# Autodesk Inventor assembly: SR-092.5-DPY
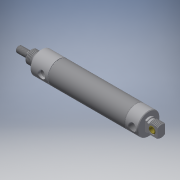
[picture p0: Inventor's stored thumbnail of the model, 180x180]
Saved by Autodesk Inventor 2016 SP1 (Build 200210100, 210)
## iProperties
Category: PARTsolutions
Company: BIMBA
Created: 2017-03-09
Part Number: SR-092.5-DPY
Catalog Web Link: www.cadenas.de
Description: Original Line Standard Air Cylinders-
Vendor: BIMBA
Document SubType Name: Assembly
Designer: 589013
Manufacturer: BIMBA
PSOL_IDENT_0: {$CADENAS_DATA\23d-libs\bimba\bimba\bimba_imperial\bimba_full_line\original_line_cylinders\standard_
PSOL_IDENT_1: air_cylinders\standard_air_cylinder_asmtab.prj},324 {VTYP=3D},{STYP=ASSTAB},{NB=SR-092.5-DPY},{LINA=
PSOL_IDENT_2: SR-092.5-DPY},{NN=Original Line Standard Air Cylinders},{DATE=09.11.2016 07:55:11},{GEOMDATE=11.07.2
PSOL_IDENT_3: 016 10:37:18},{VERSION=},{LINEID=10},{LINESUBID=-1},{WBVAR=STROKE,ACTING,MNT,DER,NR,BM,CO,OO,VO,M,EE
PSOL_IDENT_4: ,EEL,K,Q,Y,G,T,B,H,SER,SR,NT,W,HL,STPT1,STPT2,STPT3,STPT4,MB,PB,PRC,TB,MN}  {NB=SR-092.5-DPY},{LINA=
PSOL_IDENT_5: SR-092.5-DPY},{KT=DUMMY},{PN=SR-092.5-DPY},{PNC=SR-092.5-DPY},{PNA=(NO ACCESSORIES)},{DASH=-},{BORE1=
PSOL_IDENT_6: 1.06250000},{BORE=1 1/16\" (09)},{BOREPN=09},{STROKE=2.500},{STROKEALG=[0.011:50/0.001]},{STROKE1=2.
PSOL_IDENT_7: 500},{ACTING=D},{ACTINGALG= '' , 'Single Acting (SA)' , 'R' , 'Reverse Single Acting (SA)' , 'D' , '
PSOL_IDENT_8: Double Acting (SA)' },{ACTINGPN=D},{MNT=P},{MNTALG= '' , 'Front Nose Mounting (SA)' , 'P' , 'Rear Pi
PSOL_IDENT_9: vot Mounting (SA)' , 'X' , 'Universal Pivot Mounting or Double End Mounting (SA)' , 'BF' , 'Front Bl
PSOL_IDENT_10: ock Mounting (SA)' , 'BR' , 'Rear Block Mounting for Vertical Positioning (SA)' , 'BFT' , 'Front Blo
PSOL_IDENT_11: ck Trunnion Mounting (SA)' , 'BRT' , 'Rear Block Trunnion Mounting (SA)' },{TYPE=SR-},{MNTPN=P},{DER=
PSOL_IDENT_12: },{DERALG= '' , 'N/A' },{NR=},{NRALG= '' , 'N/A' },{NRPN=},{BM=},{BMALG= '' , 'N/A' },{BMPN=},{CO=},
PSOL_IDENT_13: {COALG= '' , 'N/A' },{OO=},{OOALG= '', 'N/A' },{OOPN=},{VO=Z},{VOALG= 'Z' , 'N/A' },{VOPN=},{OOVOPN=
PSOL_IDENT_14: },{M=},{MALG= '', 'Without Magnet', 'M', 'With Magnet' },{EE=},{EEL=0.000},{EEMAX=47.5000},{EEALG= ''
PSOL_IDENT_15: , 'Without Extra Extension', 'EE', 'With Extra Extension' },{EELALG=0},{EEPN=},{EEPN1=0.000},{K=},{K
PSOL_IDENT_16: ALG= '', 'Standard' , 'K' , 'Ports Rotated 90deg K' },{KPN=},{Q=},{QALG= '' , 'N/A' },{QPN=},{Y=Y},{
PSOL_IDENT_17: YALG= '' , 'Without Pivot Bushing' , 'Y' , 'With Pivot Bushing' },{YPN=Y},{YCON=Y},{F=},{FALG= '', '
PSOL_IDENT_18: Non-Coated (Standard)', 'F', 'Molycoated' },{FPN=},{G=},{GPN=},{GPN99=},{T=},{TALG= '' , 'Standard -
PSOL_IDENT_19: 20° to 200°F (-29° to 95°C)' , 'N' , 'Low Temperature' , 'V' , 'High Temperature' },{NPN=},{VPN=},{B=
PSOL_IDENT_20: },{BALG= '', 'W/out Bumpers' , 'B' , 'W/ Bumpers' },{BPN=},{H=},{HALG= '', 'N/A' },{HPN=},{SER=},{SE
PSOL_IDENT_21: RALG= '' , 'Without Spring Extend/Return' , 'JS' , 'With Spring Return' , 'JR' , 'With Spring Extend'
PSOL_IDENT_22: },{SR=SR},{SRALG= 'C' , 'Standard Blackened Carbon Steel' , 'SR' , 'Stainless Steel [SR]' },{SRPN=S
PSOL_IDENT_23: R},{SRCON=1},{NT=},{NTPN=},{W=},{WALG= '' , 'Without Wiper' , 'W' , 'With Wiper' },{WPN=},{E=},{EALG=
PSOL_IDENT_24: '' , 'Standard Seals/Lube' , 'E' , 'Non-Lube Seals/Lube' },{EPN=},{HL=},{HLALG= '' , 'Without Low P
PSOL_IDENT_25: ressure Hydraulic' , 'HL' , 'With Low Pressure Hydraulic' },{ST=},{STALG= '' , 'N/A' },{STPT1=},{STP
PSOL_IDENT_26: T1ALG= '' , 'N/A' },{STPT2=},{STPT2ALG= '' , 'N/A' },{STPT3=},{STPT3ALG= '' , 'N/A' },{STPT4=},{STPT
PSOL_IDENT_27: 4ALG= '' , 'N/A' },{STPN=},{MB=},{MBALG= '' , 'N/A' },{MBPN=},{MBPNALL=},{MBPNALLREAR=},{PB=},{PBALG=
PSOL_IDENT_28: '' , 'Without Pivot Bracket' , 'D-13498-A' , 'D-13498-A' },{PBPN=},{PBPNALL=D-13498-A},{PRC=},{PRCA
PSOL_IDENT_29: LG= '' , 'W/out Pivot Rod Clevis' , 'F,D-166-1' , 'D-166-1 (front)' },{PRCPN=},{PRCPNALL=D-166-1},{T
PSOL_IDENT_30: B=},{TBALG= '' , 'N/A' },{TBPN=},{TBPNALL=},{MN=},{MNALG= '' , 'Without Mounting Nut' , 'F,D-9' , 'D
PSOL_IDENT_31: -9 (front)' , 'R,D-9' , 'D-9 (rear)', '2x,D-9' , 'D-9 (front & rear)' },{MNPN=},{MNCONF=},{MNCONR=},
PSOL_IDENT_32: {TLEN=3.8185},{FRAC=10.8400},{RGCON=},{RGDACCON=R},{RHCON=P},{RHCON1=P},{RHCONON=1},{RHACCON=},{FNUT
PSOL_IDENT_33: CON=0},{RNUTCON=0},{FNUTPN=D-9},{RNUTPN=D-9},{FNUTTRANS=0.0000},{RNUTTRANS=0.0000},{VHOLECON=0},{A1=
PSOL_IDENT_34: 1.6250},{A1N=1.0000},{A1P=1.6250},{A1B=1.8750},{A4=0.2525},{A4N=0.3750},{A4P=0.2525},{A5=0.0300},{A1
PSOL_IDENT_35: H=1.5},{A1NH=0.6250},{A1PH=1.5000},{A1BH=1.1250},{A1SH=1.1250},{A2H=0.2500},{A2NH=0.2500},{LENGTH=3.
PSOL_IDENT_36: 8400},{LENGTH1=3.8400},{LENGTH2=4.1000},{MUL=2.5000},{MUL11=2.5000},{MUL22=6.4},{MUL33=3.9000},{MUL2=
PSOL_IDENT_37: 2.5000},{MUL211=2.5000},{MUL222=2.5600},{MUL233=1.5600},{SSS=5.0000},{RGLEN=1.4025},{RHLEN=0.9990},{
PSOL_IDENT_38: SSS1=3.0000},{A13=1.2190},{DIF=0.1200},{G5=0.7180},{ON=0},{SSADD=0.0000},{BADD=0.0000},{MADD=0.0000}
PSOL_IDENT_39: ,{NVADD=0.0000},{TRACKL=3.5285},{TRACKCON=D-78527},{TRIMCON=0},{TRIMCON1=0},{PINCON=},{FSPACE=0.7678
PSOL_IDENT_40: },{SPACE=0.0987},{TEXT=0.1727},{S1=1.2500},{D1=1.1410},{D1N=1.1130},{D1B=1.1130},{D1P=1.1410},{FA=0.
PSOL_IDENT_41: 940},{RA=0.9400},{PPATH=standard_air_cylinder_asmtpl.prj},{MATALGHTML=<b>Standard Original Line:</b>
PSOL_IDENT_42: <dl><dt>Rod:</dt><dd>- Stainless Steel</dd><dd>&nbsp;&nbsp;(5/16 9/16 Bores)</dd><dd>- High Strength
PSOL_IDENT_43: Carbon Steel</dd><dd>&nbsp;&nbsp;(3/4 3 Bore)</dd><dd>- Stainless Steel</dd><dd>&nbsp;&nbsp;(X styl
PSOL_IDENT_44: e DXP/DX/DXDE)</dd><dt>Bearings:</dt><dd>- Sintered Bronze</dd><dt>Body:</dt><dd>- 304 Stainless Ste
PSOL_IDENT_45: el</dd><dt>End Caps:</dt><dd>- Aluminum</dd><dt>Seals:</dt><dd>- Buna N</dd></dl>},{ASSCFGPRA=09DP},
PSOL_IDENT_46: {MBPNA=},{MNPNA=},{PRCPNA=},{ASSOPTACC=STPT4},{A=6.34},{HADD=0.0000},{WFL=0.125},{QADD=0.000},{QADD1=
PSOL_IDENT_47: 0.250},{TEST=2.0000},{MNTB=},{STDNUTF=0},{STDNUTR=0},{STRK2D=0},{X2D=2},{STROKESW=2.500},{EESW=0.000
PSOL_IDENT_48: },{FCD=0},{BCD=0},{RCD=0},{CUSTADD=1.500},{FT=5/16-24 UNF-2A},{FT1=5/16-24 UNF-2A},{FT2=5/8-18 UNF-2
PSOL_IDENT_49: A},{PORT=1/8 NPT},{FT11=5/8-18 UNF-2A},{FT12=5/8-18 UNF-2A}
NN: Original Line Standard Air Cylinders
NT: Standard Male Thread
NB: SR-092.5-DPY
NBSYN: $PNC.
LINA: SR-092.5-DPY
PN: SR-092.5-DPY
PNA: (NO ACCESSORIES)
BORE: 1 1/16" [09]
STROKE: 2.500
ACTING: Double [D]
MNT: Rear Pivot [P]
DER: N/A
NR: N/A
BM: N/A
CO: N/A
OO: N/A
VO: N/A
M: Without Magnet Piston
EE: Standard Rod Extension
EEL: 0.000
K: Standard
Q: N/A
Y: Pivot Bushing [Y]
G: Standard Grease Lube
T: Standard -20° to 200°F (-29° to 95°C)
B: Without Bumpers
H: N/A
SER: Without Failsafe Spring Extend/Return
SR: Stainless Steel [SR]
W: Without Wiper
HL: Standard 250 PSI Air
STPT1: N/A
STPT2: N/A
STPT3: N/A
STPT4: N/A
MB: N/A
PB: Without Pivot Bracket
PRC: Without Piston Rod Clevis
TB: N/A
MN: Without Mounting Nut
A: 6.34
SUPPLIER: BIMBA
ARTICLENO: SR-092.5-DPY
BOMINFO: SR-092.5-DPY
CREATOR: CADENAS GmbH
Title: SR-092.5-DPY
Author: Cadenas PARTsolutions
## Documents named in this file (7)
- C:\Users\589013\Downloads\SR-092_5-DPY.iam
- C:\Users\589013\Downloads\SR-092_5-DPSRY0000_0_dummy.ipt
- C:\Users\589013\Downloads\09R000-0_rod_guide.ipt
- C:\Users\589013\Downloads\09R-3_81350SR.ipt
- C:\Users\589013\Downloads\09P0Y000_rear_head.ipt
- C:\Users\589013\Downloads\D-3543.ipt
- C:\Users\589013\Downloads\SR-092_5-DPY0_rod.ipt
## Components (6 placed, 6 different names)
1. SR-092_5-DPSRY0000_0_dummy:1 — dummy_XY@1 <-> rod_guide_XY@2, dummy_Z@1 <-> rod_guide_Z@2, dummy_YZ@1 <-> rod_guide_YZ@2
2. 09R000-0_rod_guide:1 — dummy_XY@1 <-> rod_guide_XY@2, dummy_Z@1 <-> rod_guide_Z@2, dummy_YZ@1 <-> rod_guide_YZ@2, to_tube_XY@2 <-> tube_front_XY@3, to_tube_Z@2 <-> tube_front_Z@3, to_tube_YZ@2 <-> tube_front_YZ@3, to_rod_XY@2 <-> rod_cp_XY@6, to_rod_Z@2 <-> rod_cp_Z@6
3. 09R-3_81350SR:1 — to_tube_XY@2 <-> tube_front_XY@3, to_tube_Z@2 <-> tube_front_Z@3, to_tube_YZ@2 <-> tube_front_YZ@3, tube_rear_XY@3 <-> to_tube_XY@4, tube_rear_Z@3 <-> to_tube_Z@4, tube_rear_YZ@3 <-> to_tube_YZ@4
4. 09P0Y000_rear_head:1 — tube_rear_XY@3 <-> to_tube_XY@4, tube_rear_Z@3 <-> to_tube_Z@4, tube_rear_YZ@3 <-> to_tube_YZ@4, to_pin_XY@4 <-> bushing_XY@5, to_pin_Z@4 <-> bushing_Z@5, to_pin_YZ@4 <-> bushing_YZ@5
5. D-3543:1 — to_pin_XY@4 <-> bushing_XY@5, to_pin_Z@4 <-> bushing_Z@5, to_pin_YZ@4 <-> bushing_YZ@5
6. SR-092_5-DPY0_rod:1 — to_rod_XY@2 <-> rod_cp_XY@6, to_rod_Z@2 <-> rod_cp_Z@6
## Relationships (14: Mate 6, Flush 4, Angle 4)
- dummy_XY@1 <-> rod_guide_XY@2 [Flush]: SR-092_5-DPSRY0000_0_dummy:1 ↔ 09R000-0_rod_guide:1
- dummy_Z@1 <-> rod_guide_Z@2 [Mate]: SR-092_5-DPSRY0000_0_dummy:1 ↔ 09R000-0_rod_guide:1
- dummy_YZ@1 <-> rod_guide_YZ@2 [Angle] (0 deg): SR-092_5-DPSRY0000_0_dummy:1 ↔ 09R000-0_rod_guide:1
- to_tube_XY@2 <-> tube_front_XY@3 [Flush]: 09R000-0_rod_guide:1 ↔ 09R-3_81350SR:1
- to_tube_Z@2 <-> tube_front_Z@3 [Mate]: 09R000-0_rod_guide:1 ↔ 09R-3_81350SR:1
- to_tube_YZ@2 <-> tube_front_YZ@3 [Angle] (0 deg): 09R000-0_rod_guide:1 ↔ 09R-3_81350SR:1
- tube_rear_XY@3 <-> to_tube_XY@4 [Flush]: 09R-3_81350SR:1 ↔ 09P0Y000_rear_head:1
- tube_rear_Z@3 <-> to_tube_Z@4 [Mate]: 09R-3_81350SR:1 ↔ 09P0Y000_rear_head:1
- tube_rear_YZ@3 <-> to_tube_YZ@4 [Angle] (0 deg): 09R-3_81350SR:1 ↔ 09P0Y000_rear_head:1
- to_pin_XY@4 <-> bushing_XY@5 [Mate]: 09P0Y000_rear_head:1 ↔ D-3543:1
- to_pin_Z@4 <-> bushing_Z@5 [Mate]: 09P0Y000_rear_head:1 ↔ D-3543:1
- to_pin_YZ@4 <-> bushing_YZ@5 [Angle] (0 deg): 09P0Y000_rear_head:1 ↔ D-3543:1
- to_rod_XY@2 <-> rod_cp_XY@6 [Flush]: 09R000-0_rod_guide:1 ↔ SR-092_5-DPY0_rod:1
- to_rod_Z@2 <-> rod_cp_Z@6 [Mate]: 09R000-0_rod_guide:1 ↔ SR-092_5-DPY0_rod:1
